# Autodesk Inventor assembly: Робот в сборе
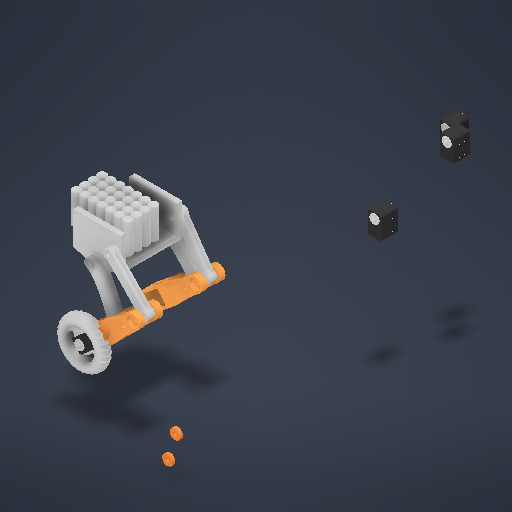
[picture p0: Inventor's stored thumbnail of the model, 512x512]
Saved by Autodesk Inventor 2025 (Build 290162010, 162A)
## iProperties
Created: 2024-06-14
Part Number: Робот в сборе
Document SubType Name: Assembly
Designer: Edward_Higgins
Author: Edward_Higgins
## Documents named in this file (9)
- D:\Users\Edward_Higgins\Desktop\ZAVOD\Робот Сколково\Робот в сборе.iam
- D:\Users\Edward_Higgins\Desktop\ZAVOD\Робот Сколково\Корпус.ipt
- D:\Users\Edward_Higgins\Desktop\ZAVOD\Робот Сколково\Нога.ipt
- D:\Users\Edward_Higgins\Desktop\ZAVOD\Робот Сколково\Тяга задняя.ipt
- D:\Users\Edward_Higgins\Desktop\ZAVOD\Робот Сколково\Тяга передняя.ipt
- D:\Users\Edward_Higgins\Desktop\ZAVOD\Робот Сколково\Подшипник.ipt
- D:\Users\Edward_Higgins\Desktop\ZAVOD\Робот Сколково\Колесо.ipt
- D:\Users\Edward_Higgins\Desktop\ZAVOD\Робот Сколково\Батарея.ipt
- D:\Users\Edward_Higgins\Desktop\ZAVOD\Робот Сколково\DYNAMIXEL XM430-W350.ipt
## Components (17 placed, 8 different names)
1. Корпус:1 — Совмещение:1, Совмещение:2, Совмещение:3, Совмещение:5, Совмещение:6, Совмещение:15, Совмещение:17, Совмещение:18, Совмещение:27
2. Нога:1 — Совмещение:7, Совмещение:22, Совмещение:24, Совмещение:25
3. Тяга задняя:1 — Совмещение:3, Совмещение:5, Совмещение:7
4. Тяга передняя:1 — Совмещение:6
5. Нога:2 — Совмещение:26, Совмещение:28
6. Тяга задняя:2 — Совмещение:15, Совмещение:17, Совмещение:28
7. Тяга передняя:2 — Совмещение:18, Совмещение:26, Совмещение:27
8. Подшипник:1
9. Подшипник:2
10. Подшипник:3
11. Подшипник:4
12. Колесо:1 — Совмещение:22, Совмещение:23
13. Батарея:1
14. DYNAMIXEL XM430-W350:1
15. DYNAMIXEL XM430-W350:2
16. DYNAMIXEL XM430-W350:3
17. DYNAMIXEL XM430-W350:4 — Совмещение:23, Совмещение:24, Совмещение:25
## Relationships (17: Mate 17)
- Совмещение:1 [Mate]: Корпус:1
- Совмещение:2 [Mate]: Корпус:1
- Совмещение:3 [Mate]: Корпус:1 ↔ Тяга задняя:1
- Совмещение:5 [Mate]: Корпус:1 ↔ Тяга задняя:1
- Совмещение:6 [Mate]: Корпус:1 ↔ Тяга передняя:1
- Совмещение:7 [Mate]: Нога:1 ↔ Тяга задняя:1
- [Mate]: Нога:2 ↔ Тяга задняя:2
- Совмещение:15 [Mate]: Корпус:1 ↔ Тяга задняя:2
- Совмещение:17 [Mate]: Корпус:1 ↔ Тяга задняя:2
- Совмещение:18 [Mate]: Корпус:1 ↔ Тяга передняя:2
- Совмещение:22 [Mate]: Нога:1 ↔ Колесо:1
- Совмещение:23 [Mate]: Колесо:1 ↔ DYNAMIXEL XM430-W350:4
- Совмещение:24 [Mate]: Нога:1 ↔ DYNAMIXEL XM430-W350:4
- Совмещение:25 [Mate]: Нога:1 ↔ DYNAMIXEL XM430-W350:4
- Совмещение:26 [Mate]: Нога:2 ↔ Тяга передняя:2
- Совмещение:27 [Mate]: Корпус:1 ↔ Тяга передняя:2
- Совмещение:28 [Mate]: Нога:2 ↔ Тяга задняя:2
## Named parameters: d10_d6 = 0 mm
